# Autodesk Inventor assembly: Babka
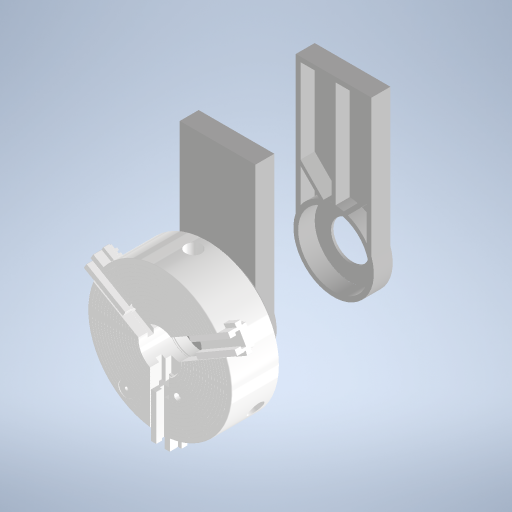
[picture p0: Inventor's stored thumbnail of the model, 512x512]
Saved by Autodesk Inventor 2024 (Build 280153000, 153)
## iProperties
Created: 2023-08-16
Part Number: Babka
Document SubType Name: Assembly
Designer: Kippi
Author: Kippi
## Documents named in this file (4)
- C:\WorkProject\CNC_Lathe\Babka.iam
- C:\WorkProject\CNC_Lathe\FlanecPodsipnikForwardBabka.ipt
- C:\WorkProject\CNC_Lathe\Rails\3 JAW CHUCK SCROLL SLIDES REAR PLATE.ipt
- C:\WorkProject\CNC_Lathe\ShaibaNaPatron.ipt
## Components (4 placed, 3 different names)
1. FlanecPodsipnikForwardBabka:1 — Flush:3, Flush:4
2. 3 JAW CHUCK SCROLL SLIDES REAR PLATE:1 — Mate:3, Mate:4
3. ShaibaNaPatron:1 — Mate:3, Mate:4
4. FlanecPodsipnikForwardBabka:3 — Flush:3, Flush:4
## Relationships (4: Mate 2, Flush 2)
- Mate:3: 3 JAW CHUCK SCROLL SLIDES REAR PLATE:1 ↔ ShaibaNaPatron:1
- Mate:4: 3 JAW CHUCK SCROLL SLIDES REAR PLATE:1 ↔ ShaibaNaPatron:1
- Flush:3: FlanecPodsipnikForwardBabka:1 ↔ FlanecPodsipnikForwardBabka:3
- Flush:4: FlanecPodsipnikForwardBabka:1 ↔ FlanecPodsipnikForwardBabka:3
